# Autodesk Inventor assembly: base_ass_2
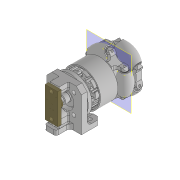
[picture p0: Inventor's stored thumbnail of the model, 180x180]
Saved by Autodesk Inventor 2020 (Build 240168000, 168)
## iProperties
Created: 2022-01-21
Part Number: base_ass_2
Document SubType Name: Assembly
Designer: Shuang Peng
Author: Shuang Peng
## Documents named in this file (5)
- D:\projects-3\soft module robot\hardware\diff module 3\base_ass_2.iam
- D:\projects-3\soft module robot\hardware\diff module 3\motor_1613_3.iam
- D:\projects-3\soft module robot\hardware\diff module 3\motor_hl_2.ipt
- D:\projects-3\soft module robot\hardware\diff module 3\ma_3.3_2_2.ipt
- D:\projects-3\soft module robot\hardware\diff module 3\Board.ipt
## Components (4 placed, 4 different names)
1. motor_1613_3:1 [sub-assembly] — Insert:6, Insert:7, Insert:8
2. motor_hl_2:1 — Insert:6, Insert:7, Angle:1
3. ma_3.3_2_2:1 — Insert:8, Insert:9
4. Board:1 — Insert:9, Angle:1
## Relationships (5: Insert 4, Angle 1)
- Insert:6: motor_1613_3:1 ↔ motor_hl_2:1
- Insert:7: motor_1613_3:1 ↔ motor_hl_2:1
- Insert:8: motor_1613_3:1 ↔ ma_3.3_2_2:1
- Insert:9 (1.5 mm): ma_3.3_2_2:1 ↔ Board:1
- Angle:1 (0 deg): motor_hl_2:1 ↔ Board:1
